# Autodesk Inventor assembly: KB33-046-003 - Рама центральная
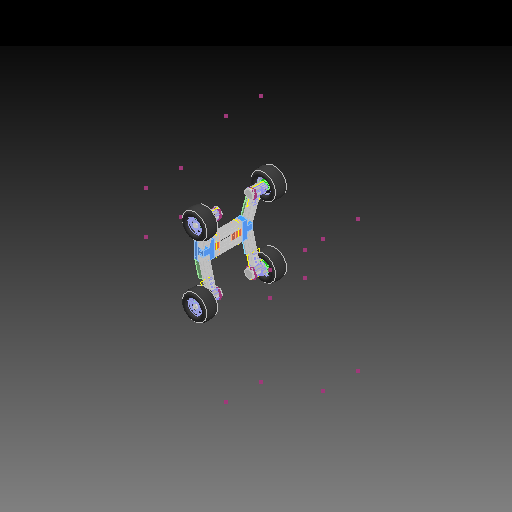
[picture p0: Inventor's stored thumbnail of the model, 512x512]
Saved by Autodesk Inventor 2020 (Build 240168000, 168)
## iProperties
Created: 2021-06-22
Part Number: KB33-046-003 - Рама центральная
Document SubType Name: Assembly
Designer: Петров Иван
Mass: 5764.24 g
Surface Area: 10888.1 cm^2
Volume: 5700.89 cm^3
Density: 1.01111 g/cm^3
Author: Петров Иван
## Documents named in this file (8)
- E:\IVAN\Ivan_desktop\Kvantorium\Projects\RoboPatrol\design\KB33-046-003 - Рама центральная.iam
- E:\IVAN\Ivan_desktop\Kvantorium\Projects\RoboPatrol\design\standart_components\Tetrix\ftc-tetrix-kit-of-parts-1.snapshot.34\MAX Channels\160mm Channel.ipt
- E:\IVAN\Ivan_desktop\Kvantorium\Projects\RoboPatrol\design\KB33-046-003-001 - Соединитель.ipt
- E:\IVAN\Ivan_desktop\Kvantorium\Projects\RoboPatrol\design\KB33-046-003-002 - Кожух рычагов.ipt
- E:\IVAN\Ivan_desktop\Kvantorium\Projects\RoboPatrol\design\KB33-046-003-003 - Накладка на рычаг.ipt
- E:\IVAN\Ivan_desktop\Kvantorium\Projects\RoboPatrol\design\KB33-046-003-003 - Накладка на рычаг зеркальный.ipt
- E:\IVAN\Ivan_desktop\Kvantorium\Projects\RoboPatrol\design\KB33-046-002 - Привод в сборе.iam
- E:\IVAN\Ivan_desktop\Kvantorium\Projects\RoboPatrol\design\KB33-046-002 - Привод в сборе зеркальный.iam
## Components (18 placed, 7 different names)
1. 160mm Channel:1 — Совмещение:1, Заподлицо:1, Заподлицо:2, Угол:2, Совмещение:10, Заподлицо:4, Совмещение:16
2. 160mm Channel:2 — Совмещение:1, Заподлицо:1, Заподлицо:2, Угол:1, Совмещение:4, Совмещение:5, Заподлицо:3, Совмещение:9
3. 160mm Channel:3 — Угол:1, Совмещение:6, Заподлицо:5, Совмещение:23, Совмещение:28, Совмещение:29, Совмещение:44, Совмещение:53, Совмещение:54, Совмещение:55
4. KB33-046-003-001 - Соединитель:1 — Совмещение:4, Совмещение:5, Заподлицо:3, Совмещение:6, Совмещение:8, Совмещение:42
5. 160mm Channel:4 — Совмещение:8, Угол:2, Заподлицо:6, Совмещение:25, Совмещение:26, Совмещение:36, Совмещение:37, Совмещение:38, Совмещение:43
6. 160mm Channel:5 — Заподлицо:5, Совмещение:20, Совмещение:39, Совмещение:40, Совмещение:41, Совмещение:46, Совмещение:47
7. KB33-046-003-001 - Соединитель:2 — Совмещение:9, Совмещение:10, Заподлицо:4, Совмещение:17, Совмещение:45
8. 160mm Channel:6 — Заподлицо:6, Совмещение:30, Совмещение:32, Совмещение:48, Совмещение:49, Совмещение:50, Совмещение:51, Совмещение:52
9. KB33-046-003-002 - Кожух рычагов:1 — Совмещение:16, Совмещение:17, Заподлицо:7, Совмещение:21, Заподлицо:8, Совмещение:31, Совмещение:45, Совмещение:46, Совмещение:47, Совмещение:48, Совмещение:49
10. KB33-046-003-002 - Кожух рычагов:2 — Заподлицо:7, Совмещение:23, Совмещение:24, Совмещение:27, Совмещение:42, Совмещение:43, Совмещение:44
11. KB33-046-003-003 - Накладка на рычаг:1 — Совмещение:20, Совмещение:21, Заподлицо:8
12. KB33-046-003-003 - Накладка на рычаг:2 — Совмещение:24, Совмещение:25, Совмещение:26
13. KB33-046-003-003 - Накладка на рычаг зеркальный:1 — Совмещение:30, Совмещение:31, Совмещение:32
14. KB33-046-003-003 - Накладка на рычаг зеркальный:2 — Совмещение:27, Совмещение:28, Совмещение:29
15. KB33-046-002 - Привод в сборе:2 [sub-assembly] — Совмещение:36, Совмещение:37, Совмещение:38
16. KB33-046-002 - Привод в сборе:3 [sub-assembly] — Совмещение:39, Совмещение:40, Совмещение:41
17. KB33-046-002 - Привод в сборе зеркальный:1 [sub-assembly] — Совмещение:50, Совмещение:51, Совмещение:52
18. KB33-046-002 - Привод в сборе зеркальный:2 [sub-assembly] — Совмещение:53, Совмещение:54, Совмещение:55
## Relationships (51: Mate 41, Flush 8, Angle 2)
- Совмещение:1 [Mate] (40 mm): 160mm Channel:1 ↔ 160mm Channel:2
- Заподлицо:1 [Flush]: 160mm Channel:1 ↔ 160mm Channel:2
- Заподлицо:2 [Flush]: 160mm Channel:1 ↔ 160mm Channel:2
- Угол:1 [Angle] (-15 deg): 160mm Channel:2 ↔ 160mm Channel:3
- Совмещение:4 [Mate]: 160mm Channel:2 ↔ KB33-046-003-001 - Соединитель:1
- Совмещение:5 [Mate]: 160mm Channel:2 ↔ KB33-046-003-001 - Соединитель:1
- Заподлицо:3 [Flush]: 160mm Channel:2 ↔ KB33-046-003-001 - Соединитель:1
- Совмещение:6 [Mate]: 160mm Channel:3 ↔ KB33-046-003-001 - Соединитель:1
- Совмещение:8 [Mate]: KB33-046-003-001 - Соединитель:1 ↔ 160mm Channel:4
- Угол:2 [Angle] (15 deg): 160mm Channel:1 ↔ 160mm Channel:4
- Совмещение:9 [Mate]: 160mm Channel:2 ↔ KB33-046-003-001 - Соединитель:2
- Совмещение:10 [Mate]: 160mm Channel:1 ↔ KB33-046-003-001 - Соединитель:2
- Заподлицо:4 [Flush]: 160mm Channel:1 ↔ KB33-046-003-001 - Соединитель:2
- Заподлицо:5 [Flush]: 160mm Channel:3 ↔ 160mm Channel:5
- Заподлицо:6 [Flush]: 160mm Channel:4 ↔ 160mm Channel:6
- Совмещение:16 [Mate]: 160mm Channel:1 ↔ KB33-046-003-002 - Кожух рычагов:1
- Совмещение:17 [Mate]: KB33-046-003-001 - Соединитель:2 ↔ KB33-046-003-002 - Кожух рычагов:1
- Заподлицо:7 [Flush]: KB33-046-003-002 - Кожух рычагов:1 ↔ KB33-046-003-002 - Кожух рычагов:2
- Совмещение:20 [Mate]: 160mm Channel:5 ↔ KB33-046-003-003 - Накладка на рычаг:1
- Совмещение:21 [Mate]: KB33-046-003-002 - Кожух рычагов:1 ↔ KB33-046-003-003 - Накладка на рычаг:1
- Заподлицо:8 [Flush] (2.5 mm): KB33-046-003-002 - Кожух рычагов:1 ↔ KB33-046-003-003 - Накладка на рычаг:1
- Совмещение:23 [Mate]: 160mm Channel:3 ↔ KB33-046-003-002 - Кожух рычагов:2
- Совмещение:24 [Mate]: KB33-046-003-002 - Кожух рычагов:2 ↔ KB33-046-003-003 - Накладка на рычаг:2
- Совмещение:25 [Mate]: 160mm Channel:4 ↔ KB33-046-003-003 - Накладка на рычаг:2
- Совмещение:26 [Mate]: 160mm Channel:4 ↔ KB33-046-003-003 - Накладка на рычаг:2
- Совмещение:27 [Mate]: KB33-046-003-002 - Кожух рычагов:2 ↔ KB33-046-003-003 - Накладка на рычаг зеркальный:2
- Совмещение:28 [Mate]: 160mm Channel:3 ↔ KB33-046-003-003 - Накладка на рычаг зеркальный:2
- Совмещение:29 [Mate]: 160mm Channel:3 ↔ KB33-046-003-003 - Накладка на рычаг зеркальный:2
- Совмещение:30 [Mate]: 160mm Channel:6 ↔ KB33-046-003-003 - Накладка на рычаг зеркальный:1
- Совмещение:31 [Mate]: KB33-046-003-002 - Кожух рычагов:1 ↔ KB33-046-003-003 - Накладка на рычаг зеркальный:1
- Совмещение:32 [Mate]: 160mm Channel:6 ↔ KB33-046-003-003 - Накладка на рычаг зеркальный:1
- Совмещение:36 [Mate]: 160mm Channel:4 ↔ KB33-046-002 - Привод в сборе:2
- Совмещение:37 [Mate]: 160mm Channel:4 ↔ KB33-046-002 - Привод в сборе:2
- Совмещение:38 [Mate]: 160mm Channel:4 ↔ KB33-046-002 - Привод в сборе:2
- Совмещение:39 [Mate]: 160mm Channel:5 ↔ KB33-046-002 - Привод в сборе:3
- Совмещение:40 [Mate]: 160mm Channel:5 ↔ KB33-046-002 - Привод в сборе:3
- Совмещение:41 [Mate]: 160mm Channel:5 ↔ KB33-046-002 - Привод в сборе:3
- Совмещение:42 [Mate]: KB33-046-003-001 - Соединитель:1 ↔ KB33-046-003-002 - Кожух рычагов:2
- Совмещение:43 [Mate]: 160mm Channel:4 ↔ KB33-046-003-002 - Кожух рычагов:2
- Совмещение:44 [Mate]: 160mm Channel:3 ↔ KB33-046-003-002 - Кожух рычагов:2
- Совмещение:45 [Mate]: KB33-046-003-001 - Соединитель:2 ↔ KB33-046-003-002 - Кожух рычагов:1
- Совмещение:46 [Mate]: 160mm Channel:5 ↔ KB33-046-003-002 - Кожух рычагов:1
- Совмещение:47 [Mate]: 160mm Channel:5 ↔ KB33-046-003-002 - Кожух рычагов:1
- Совмещение:48 [Mate]: 160mm Channel:6 ↔ KB33-046-003-002 - Кожух рычагов:1
- Совмещение:49 [Mate]: 160mm Channel:6 ↔ KB33-046-003-002 - Кожух рычагов:1
- Совмещение:50 [Mate]: 160mm Channel:6 ↔ KB33-046-002 - Привод в сборе зеркальный:1
- Совмещение:51 [Mate]: 160mm Channel:6 ↔ KB33-046-002 - Привод в сборе зеркальный:1
- Совмещение:52 [Mate]: 160mm Channel:6 ↔ KB33-046-002 - Привод в сборе зеркальный:1
- Совмещение:53 [Mate]: 160mm Channel:3 ↔ KB33-046-002 - Привод в сборе зеркальный:2
- Совмещение:54 [Mate]: 160mm Channel:3 ↔ KB33-046-002 - Привод в сборе зеркальный:2
- Совмещение:55 [Mate]: 160mm Channel:3 ↔ KB33-046-002 - Привод в сборе зеркальный:2
